# Autodesk Inventor assembly: ASY GBK 3130 central wall shield 3
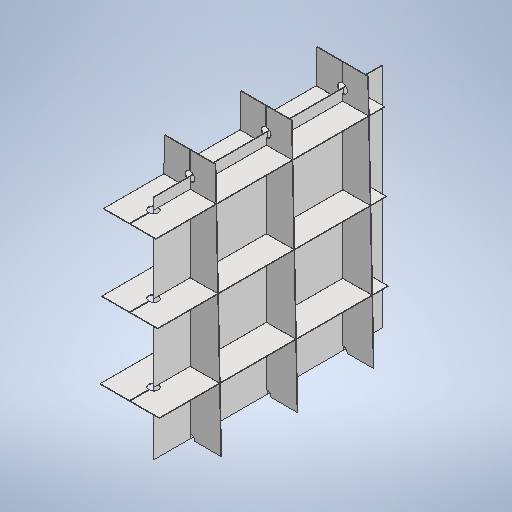
[picture p0: Inventor's stored thumbnail of the model, 512x512]
Saved by Autodesk Inventor 2026 (Build 300175000, 175)
## iProperties
Created: 2026-05-19
Part Number: ASY GBK 3130 central wall shield 3
Document SubType Name: Assembly
Designer: pokla
Mass: 174041 g
Surface Area: 113034 cm^2
Volume: 22170.8 cm^3
Density: 7.85 g/cm^3
Author: admin
## Documents named in this file (8)
- C:\Users\pokla\Documents\Inventor\GBK-Gubkinskiy\ASY GBK 3130 central wall shield 3.iam
- C:\Users\pokla\Documents\Inventor\GBK-Gubkinskiy\GBK 0101 main rib.ipt
- C:\Users\pokla\Documents\Inventor\GBK-Gubkinskiy\GBK 3133 shield 3.ipt
- C:\Users\pokla\Documents\Inventor\GBK-Gubkinskiy\GBK 3112 central main rib_CPY1.ipt
- GBK 3112 central main rib_CPY1.ipt
- C:\Users\pokla\Documents\Inventor\GBK-Gubkinskiy\GBK 3113 stringer 1.ipt
- C:\Users\pokla\Documents\Inventor\GBK-Gubkinskiy\GBK 3114 stringer 2.ipt
- C:\Users\pokla\Documents\Inventor\GBK-Gubkinskiy\GBK 3115 stringer 3.ipt
## Components (13 placed, 6 different names)
1. GBK 3113 stringer 1.ipt:1 — Жесткий:1
2. GBK 3133 shield 3.ipt:1 — Совмещение:1, Заподлицо:1, Совмещение:2, Заподлицо:3, Совмещение:5, Заподлицо:2, Совмещение:4, Заподлицо:6
3. GBK 3114 stringer 2.ipt:1 — Жесткий:2
4. GBK 3115 stringer 3.ipt:1 — Жесткий:3, Жесткий:9, Жесткий:10
5. GBK 3113 stringer 1.ipt:2 — Жесткий:6
6. GBK 3114 stringer 2.ipt:2 — Жесткий:5
7. GBK 3115 stringer 3.ipt:2 — Жесткий:6, Заподлицо:6, Жесткий:7, Жесткий:8
8. GBK 3112 central main rib_CPY1.ipt:1 — Заподлицо:3, Совмещение:5, Заподлицо:4, Жесткий:3, Жесткий:2, Жесткий:1
9. GBK 3112 central main rib_CPY1.ipt:2 — Заподлицо:2, Совмещение:4, Заподлицо:4, Жесткий:6, Жесткий:5, Жесткий:6
10. GBK 3112 central main rib_CPY1:3 — Жесткий:7
11. GBK 3112 central main rib_CPY1:4 — Жесткий:8
12. GBK 3112 central main rib_CPY1:5 — Жесткий:9
13. GBK 3112 central main rib_CPY1:6 — Жесткий:10
## Relationships (19: WeldJoint 10, Flush 5, Mate 4)
- Совмещение:1 [Mate]: GBK 3133 shield 3.ipt:1
- Заподлицо:1 [Flush]: GBK 3133 shield 3.ipt:1
- Совмещение:2 [Mate]: GBK 3133 shield 3.ipt:1
- Заподлицо:3 [Flush]: GBK 3133 shield 3.ipt:1 ↔ GBK 3112 central main rib_CPY1.ipt:1
- Совмещение:5 [Mate]: GBK 3133 shield 3.ipt:1 ↔ GBK 3112 central main rib_CPY1.ipt:1
- Заподлицо:2 [Flush]: GBK 3133 shield 3.ipt:1 ↔ GBK 3112 central main rib_CPY1.ipt:2
- Совмещение:4 [Mate]: GBK 3133 shield 3.ipt:1 ↔ GBK 3112 central main rib_CPY1.ipt:2
- Заподлицо:4 [Flush]: GBK 3112 central main rib_CPY1.ipt:1 ↔ GBK 3112 central main rib_CPY1.ipt:2
- Жесткий:3 [WeldJoint] (4 mm): GBK 3115 stringer 3.ipt:1 ↔ GBK 3112 central main rib_CPY1.ipt:1
- Жесткий:2 [WeldJoint] (4 mm): GBK 3114 stringer 2.ipt:1 ↔ GBK 3112 central main rib_CPY1.ipt:1
- Жесткий:1 [WeldJoint] (4 mm): GBK 3113 stringer 1.ipt:1 ↔ GBK 3112 central main rib_CPY1.ipt:1
- Жесткий:6 [WeldJoint] (4 mm): GBK 3113 stringer 1.ipt:2 ↔ GBK 3112 central main rib_CPY1.ipt:2
- Жесткий:5 [WeldJoint] (4 mm): GBK 3114 stringer 2.ipt:2 ↔ GBK 3112 central main rib_CPY1.ipt:2
- Жесткий:6 [WeldJoint] (4 mm): GBK 3115 stringer 3.ipt:2 ↔ GBK 3112 central main rib_CPY1.ipt:2
- Заподлицо:6 [Flush] (155 mm): GBK 3133 shield 3.ipt:1 ↔ GBK 3115 stringer 3.ipt:2
- Жесткий:7 [WeldJoint] (4 mm): GBK 3115 stringer 3.ipt:2 ↔ GBK 3112 central main rib_CPY1:3
- Жесткий:8 [WeldJoint] (4 mm): GBK 3115 stringer 3.ipt:2 ↔ GBK 3112 central main rib_CPY1:4
- Жесткий:9 [WeldJoint] (4 mm): GBK 3115 stringer 3.ipt:1 ↔ GBK 3112 central main rib_CPY1:5
- Жесткий:10 [WeldJoint] (4 mm): GBK 3115 stringer 3.ipt:1 ↔ GBK 3112 central main rib_CPY1:6
## Named parameters: основание_длина_нижнего = 200 mm, основание_длина_верхнего = 100 mm, стрингер_глубина_1 = 190.70056 mm, стрингер_глубина_2 = 179.35977 mm, стрингер_глубина_3 = 168.01899 mm, стрингер_глубина_4 = 156.6782 mm, стрингер_глубина_5 = 145.33742 mm, стрингер_глубина_6 = 133.99663 mm, стрингер_глубина_7 = 122.65585 mm, стрингер_глубина_8 = 111.31507 mm, Лист_ширина = 1480 mm, ребро_усилителей = 60 mm, паз_под_стрингер_глубина = 70 mm, паз_под_стрингер_толщина = 5 mm, отступ_от_пола_до_первого_стрингера = 410 mm, шаг_стрингеров = 500 mm, радиус_выреза_под_сварку = 30 mm, нахлест_шпангоутов_1_2 = 150 mm, нахлест_шпангоутов_2_3 = 120 mm, Стрингер_длина = 1489.5 mm, Лист_длина = 2980 mm, Шаг_шпангоутов = 496.66667 mm
